# Autodesk Inventor assembly: CLB_056_TopBarScissorWithPlug
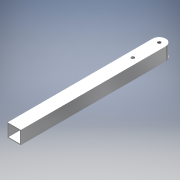
[picture p0: Inventor's stored thumbnail of the model, 180x180]
Saved by Autodesk Inventor 2018.3 (Build 223284000, 284)
## iProperties
Created: 2020-02-16
Part Number: CLB_056_TopBarScissorWithPlug
Document SubType Name: Assembly
Designer: 22perngrac
Author: 22perngrac
## Documents named in this file (3)
- C:\Users\22perngrac\Documents\GrabCAD\Infinite Recharge 2020\Build season\CLB_056_TopBarScissorWithPlug.iam
- C:\Users\22perngrac\Documents\GrabCAD\Infinite Recharge 2020\Build season\CLB_053_ScissorTopBarPlug.ipt
- C:\Users\22perngrac\Documents\GrabCAD\Infinite Recharge 2020\Build season\CLB_036_ScissorLiftBarTop.ipt
## Components (2 placed, 2 different names)
1. CLB_053_ScissorTopBarPlug:1 — Mate:1, Mate:2, Flush:1
2. CLB_036_ScissorLiftBarTop:1 — Mate:1, Mate:2, Flush:1
## Relationships (3: Mate 2, Flush 1)
- Mate:1: CLB_053_ScissorTopBarPlug:1 ↔ CLB_036_ScissorLiftBarTop:1
- Mate:2: CLB_053_ScissorTopBarPlug:1 ↔ CLB_036_ScissorLiftBarTop:1
- Flush:1 (255.5748 mm): CLB_053_ScissorTopBarPlug:1 ↔ CLB_036_ScissorLiftBarTop:1
